# Autodesk Inventor assembly: リンク_6_1
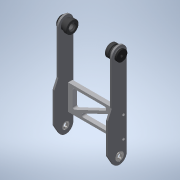
[picture p0: Inventor's stored thumbnail of the model, 180x180]
Saved by Autodesk Inventor 2020 (Build 240168000, 168)
## iProperties
Created: 2016-08-23
Part Number: リンク_6_1
Material: 一般
Document SubType Name: Assembly
Designer: hiro
Mass: 25.265 g
Surface Area: 146.992 cm^2
Volume: 11.3922 cm^3
Density: 2.21774 g/cm^3
Author: hiro
## Documents named in this file (8)
- C:\Users\Masato\Documents\Inventor\CIT Brains_Inventor\OpenPlatform_ver3_0\下半身_160823\リンク\リンク_6_3.iam
- C:\Users\Masato\Documents\Inventor\CIT Brains_Inventor\OpenPlatform_ver3_0\既製品\NSK_RB_MF85ZZ\MF85ZZ.iam
- C:\Users\Masato\Documents\Inventor\CIT Brains_Inventor\OpenPlatform_ver3_0\下半身\リンク\ふくらはぎ\リンク_ふくらはぎ_サブフレーム_1_2(予備案).ipt
- C:\Users\Masato\Documents\Inventor\CIT Brains_Inventor\OpenPlatform_ver3_0\下半身_160823\リンク\リンク_メインフレーム_6_3.ipt
- C:\Users\Masato\Documents\Inventor\CIT Brains_Inventor\OpenPlatform_ver3_0\既製品\新規購入\80F-0608.ipt
- C:\Users\Masato\Documents\Inventor\CIT Brains_Inventor\OpenPlatform_ver3_0\既製品\新規購入\GSB-081235.ipt
- C:\Users\Masato\Documents\Inventor\CIT Brains_Inventor\OpenPlatform_ver3_0\既製品\新規購入\GSB-081404.ipt
- C:\Users\Masato\Documents\Inventor\CIT Brains_Inventor\OpenPlatform_ver3_0\既製品\新規購入\FFW-0312-20B.ipt
## Components (13 placed, 7 different names)
1. MF85ZZ:1 [sub-assembly] — 挿入:9
2. MF85ZZ:2 [sub-assembly] — 挿入:10
3. リンク_ふくらはぎ_サブフレーム_1_2(予備案):1 — 挿入:2, 挿入:4, 挿入:19, 挿入:20
4. リンク_メインフレーム_6_3:1 — 挿入:2, 挿入:10, 挿入:12, 挿入:13, メイト:1, 挿入:19
5. リンク_メインフレーム_6_3:2 — 挿入:4, 挿入:9, 挿入:11, 挿入:14, 挿入:20
6. 80F-0608:1 — 挿入:11, 挿入:18
7. 80F-0608:2 — 挿入:12, 挿入:17
8. GSB-081235:1 — 挿入:13, 挿入:16
9. GSB-081235:2 — 挿入:14, 挿入:15
10. GSB-081404:1 — 挿入:15
11. GSB-081404:2 — 挿入:16
12. FFW-0312-20B:1 — 挿入:17
13. FFW-0312-20B:2 — 挿入:18
## Relationships (15: Insert 14, Mate 1)
- 挿入:2 [Insert]: リンク_ふくらはぎ_サブフレーム_1_2(予備案):1 ↔ リンク_メインフレーム_6_3:1
- 挿入:4 [Insert]: リンク_ふくらはぎ_サブフレーム_1_2(予備案):1 ↔ リンク_メインフレーム_6_3:2
- 挿入:9 [Insert]: MF85ZZ:1 ↔ リンク_メインフレーム_6_3:2
- 挿入:10 [Insert]: MF85ZZ:2 ↔ リンク_メインフレーム_6_3:1
- 挿入:11 [Insert]: リンク_メインフレーム_6_3:2 ↔ 80F-0608:1
- 挿入:12 [Insert]: リンク_メインフレーム_6_3:1 ↔ 80F-0608:2
- 挿入:13 [Insert]: リンク_メインフレーム_6_3:1 ↔ GSB-081235:1
- 挿入:14 [Insert]: リンク_メインフレーム_6_3:2 ↔ GSB-081235:2
- 挿入:15 [Insert]: GSB-081235:2 ↔ GSB-081404:1
- 挿入:16 [Insert]: GSB-081235:1 ↔ GSB-081404:2
- メイト:1 [Mate]: リンク_メインフレーム_6_3:1
- 挿入:17 [Insert]: 80F-0608:2 ↔ FFW-0312-20B:1
- 挿入:18 [Insert]: 80F-0608:1 ↔ FFW-0312-20B:2
- 挿入:19 [Insert]: リンク_ふくらはぎ_サブフレーム_1_2(予備案):1 ↔ リンク_メインフレーム_6_3:1
- 挿入:20 [Insert]: リンク_ふくらはぎ_サブフレーム_1_2(予備案):1 ↔ リンク_メインフレーム_6_3:2
